# Autodesk Inventor assembly: wheel
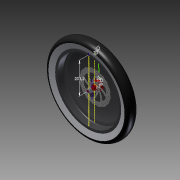
[picture p0: Inventor's stored thumbnail of the model, 180x180]
Saved by Autodesk Inventor 2014 (Build 180170000, 170)
## iProperties
Created: 2014-03-12
Part Number: wheel
Document SubType Name: Assembly
Designer: Yann
Author: Yann
## Documents named in this file (19)
- C:\Users\Yann\Documents\GitHub\BIKAIR_CAD\Source\Rear_Train\Wheel\wheel.iam
- C:\Users\Yann\Documents\GitHub\BIKAIR_CAD\Source\Rear_Train\Wheel\wheel_hub_spacer.ipt
- C:\Users\Yann\Documents\GitHub\BIKAIR_CAD\Source\Rear_Train\Wheel\wheel_rim.ipt
- C:\Users\Yann\Documents\GitHub\BIKAIR_CAD\Source\Rear_Train\Wheel\wheel_tyre.ipt
- C:\Users\Yann\Documents\GitHub\BIKAIR_CAD\Source\Rear_Train\Wheel\Disk_brake.ipt
- C:\Users\Yann\Documents\GitHub\BIKAIR_CAD\Source\Rear_Train\Wheel\Wheel_external_hub_ring.ipt
- C:\Users\Yann\Documents\GitHub\BIKAIR_CAD\Source\Rear_Train\Wheel\DIN 6912 - M5 x 40.ipt
- C:\Users\Yann\Documents\GitHub\BIKAIR_CAD\Source\Rear_Train\Wheel\ANSI B18.16.3M - M6 x 1 Type de métal.ipt
- C:\Users\Yann\Documents\GitHub\BIKAIR_CAD\Source\Rear_Train\Wheel\ANSI B18.16.3M - M14 x 2 Type de métal.ipt
- C:\Users\Yann\Documents\GitHub\BIKAIR_CAD\Source\Rear_Train\Wheel\wheel_rim_mold_A.ipt
- C:\Users\Yann\Documents\GitHub\BIKAIR_CAD\Source\Rear_Train\Wheel\wheel_rim_mold_B.ipt
- C:\Users\Yann\Documents\GitHub\BIKAIR_CAD\Source\Rear_Train\Wheel\Ground.ipt
- C:\Users\Yann\Documents\GitHub\BIKAIR_CAD\Source\Rear_Train\Wheel\wheel_rim_mold_C.ipt
- C:\Users\Yann\Documents\GitHub\Velocar_CAD\Workspaces\Espace de travail\Source\Front_train\wheel\AIP\FEA\b3969w3kw.fins
- C:\Users\Yann\Documents\GitHub\Velocar_CAD\Workspaces\Espace de travail\Source\Front_train\wheel\AIP\FEA\b3969w3kw.fsat
- C:\Users\Yann\Documents\GitHub\Velocar_CAD\Workspaces\Espace de travail\Source\Front_train\wheel\AIP\FEA\b3969w3kw.ftes
- C:\Users\Yann\Documents\GitHub\Velocar_CAD\Workspaces\Espace de travail\Source\Front_train\wheel\AIP\FEA\b3969w3kw.fwiz
- C:\Users\Yann\Documents\GitHub\Velocar_CAD\Workspaces\Espace de travail\Source\Front_train\wheel\AIP\FEA\b3969w3q8.fmsh
- C:\Users\Yann\Documents\GitHub\Velocar_CAD\Workspaces\Espace de travail\Source\Front_train\wheel\AIP\FEA\b3969w3q9.fres
## Components (17 placed, 12 different names)
1. wheel_tyre:1 — Placage:13, Placage:14, Placage:15, Tangente:1
2. wheel_hub_spacer:1 — Placage:1, Affleurement:2, Placage:2, Placage:12, Rotation:10, Rotation:11
3. wheel_rim:1 — Placage:3, Placage:4, Placage:5, Rotation:8, Affleurement:4
4. Ecrou hexagonal autofreiné à embase - Acier - Métrique M14 x 2 Type de métal:1 — Rotation:10
5. Disk_brake:1 — Rotation:11, Placage:17
6. Wheel_external_hub_ring:1 — Placage:12, Rotation:8, Rotation:12
7. wheel_rim_mold_A:1 — Affleurement:3, Affleurement:4, Affleurement:5
8. wheel_rim_mold_B:1 — Affleurement:6, Affleurement:7, Affleurement:8
9. Ground:1 — Angle:1, Tangente:1, Affleurement:9, Affleurement:10
10. Ecrou hexagonal autofreiné à embase - Acier - Métrique M6 x 1 Type de métal:1 — Placage:16, Placage:17
11. wheel_rim_mold_C:1 — Affleurement:11, Affleurement:12, Affleurement:13
12. DIN 6912 M5 x 40:1 — Placage:16, Rotation:12
13. DIN 6912 M5 x 40:2
14. DIN 6912 M5 x 40:3
15. DIN 6912 M5 x 40:4
16. DIN 6912 M5 x 40:5
17. DIN 6912 M5 x 40:6
## Component patterns: (6 elements, first: DIN 6912 M5 x 40:1)
## Relationships (29: Flush 12, Mate 11, RevoluteJoint 4, Angle 1, Tangent 1)
- Placage:1 [Mate]: wheel_hub_spacer:1
- Affleurement:2 [Flush]: wheel_hub_spacer:1
- Placage:2 [Mate]: wheel_hub_spacer:1
- Placage:3 [Mate]: wheel_rim:1
- Placage:4 [Mate]: wheel_rim:1
- Placage:5 [Mate]: wheel_rim:1
- Placage:12 [Mate]: wheel_hub_spacer:1 ↔ Wheel_external_hub_ring:1
- Rotation:8 [RevoluteJoint]: wheel_rim:1 ↔ Wheel_external_hub_ring:1
- Rotation:10 [RevoluteJoint]: wheel_hub_spacer:1 ↔ Ecrou hexagonal autofreiné à embase - Acier - Métrique M14 x 2 Type de métal:1
- Affleurement:3 [Flush]: wheel_rim_mold_A:1
- Affleurement:4 [Flush]: wheel_rim:1 ↔ wheel_rim_mold_A:1
- Affleurement:5 [Flush]: wheel_rim_mold_A:1
- Affleurement:6 [Flush]: wheel_rim_mold_B:1
- Affleurement:7 [Flush]: wheel_rim_mold_B:1
- Affleurement:8 [Flush]: wheel_rim_mold_B:1
- Angle:1 (0 deg): Ground:1
- Placage:13 [Mate]: wheel_tyre:1
- Placage:14 [Mate]: wheel_tyre:1
- Placage:15 [Mate]: wheel_tyre:1
- Tangente:1: wheel_tyre:1 ↔ Ground:1
- Affleurement:9 [Flush]: Ground:1
- Affleurement:10 [Flush]: Ground:1
- Rotation:11 [RevoluteJoint]: wheel_hub_spacer:1 ↔ Disk_brake:1
- Placage:16 [Mate]: Ecrou hexagonal autofreiné à embase - Acier - Métrique M6 x 1 Type de métal:1 ↔ DIN 6912 M5 x 40:1
- Placage:17 [Mate]: Disk_brake:1 ↔ Ecrou hexagonal autofreiné à embase - Acier - Métrique M6 x 1 Type de métal:1
- Rotation:12 [RevoluteJoint]: Wheel_external_hub_ring:1 ↔ DIN 6912 M5 x 40:1
- Affleurement:11 [Flush]: wheel_rim_mold_C:1
- Affleurement:12 [Flush]: wheel_rim_mold_C:1
- Affleurement:13 [Flush]: wheel_rim_mold_C:1
## Named parameters: sa_0 = 0, sa_1 = 0, sa_2 = -170000
note: some values were not read from the file. Shown as the stored number, unit unknown: "sa_0", "sa_1", "sa_2".
